# Autodesk Inventor assembly: bnc-nut-holder
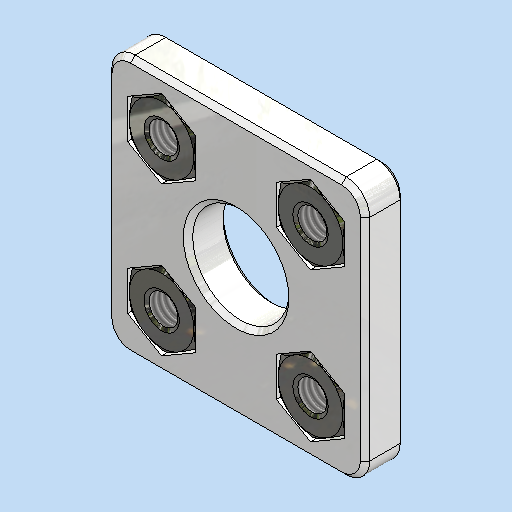
[picture p0: Inventor's stored thumbnail of the model, 512x512]
Saved by Autodesk Inventor 2025 (Build 290162000, 162)
## iProperties
Created: 2024-12-23
Part Number: bnc-nut-holder
Document SubType Name: Assembly
Designer: queezz
Author: queezz
## Documents named in this file (3)
- C:\Users\queezz\Dropbox\Drawings\PIHTI\ElectronicsBox\bnc-nut-holder.iam
- C:\Users\queezz\Dropbox\Drawings\PIHTI\ElectronicsBox\bnc-nut-support.ipt
- C:\Users\queezz\Dropbox\Drawings\PIHTI\ContentCenter\Fastners\M3-nut.ipt
## Components (5 placed, 2 different names)
1. bnc-nut-support:1
2. JIS B 1181 Style 1 - Metric A M3:1
3. JIS B 1181 Style 1 - Metric A M3:2
4. JIS B 1181 Style 1 - Metric A M3:3
5. JIS B 1181 Style 1 - Metric A M3:4
## Relationships (4: WeldJoint 4)
- [WeldJoint]: bnc-nut-support:1 ↔ JIS B 1181 Style 1 - Metric A M3:4
- [WeldJoint]: bnc-nut-support:1 ↔ JIS B 1181 Style 1 - Metric A M3:3
- [WeldJoint]: bnc-nut-support:1 ↔ JIS B 1181 Style 1 - Metric A M3:2
- [WeldJoint]: bnc-nut-support:1 ↔ JIS B 1181 Style 1 - Metric A M3:1
